# Autodesk Inventor assembly: frEonV2-AF
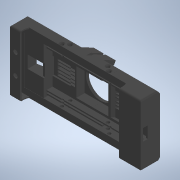
[picture p0: Inventor's stored thumbnail of the model, 180x180]
Saved by Autodesk Inventor 2020 (Build 240168000, 168)
## iProperties
Created: 2021-10-12
Part Number: frEonV2-AF
Document SubType Name: Assembly
Designer: khonsu
Author: khonsu
## Documents named in this file (5)
- D:\CAD\leeco-freon\V2\frEonV2-AF.iam
- D:\CAD\leeco-freon\V2\printed parts\left-AF.ipt
- D:\CAD\leeco-freon\V2\printed parts\right-noEONpcb-AF.ipt
- D:\CAD\leeco-freon\V2\printed parts\middle\IR-less\28DEG-CFPC-integrated.ipt
- D:\CAD\leeco-freon\V2\printed parts\middle\IR-less\bottom.ipt
## Components (4 placed, 4 different names)
1. left-AF:1 — Flush:1, Mate:1, Flush:2, Mate:3, Mate:4, Flush:3, Mate:5, Mate:6
2. right-noEONpcb-AF:1 — Flush:1, Mate:1, Flush:2, Flush:4
3. 28DEG-CFPC-integrated:1 — Mate:3, Mate:4, Flush:3
4. bottom:1 — Flush:4, Mate:5, Mate:6
## Relationships (9: Mate 5, Flush 4)
- Flush:1: left-AF:1 ↔ right-noEONpcb-AF:1
- Mate:1: left-AF:1 ↔ right-noEONpcb-AF:1
- Flush:2: left-AF:1 ↔ right-noEONpcb-AF:1
- Mate:3: left-AF:1 ↔ 28DEG-CFPC-integrated:1
- Mate:4: left-AF:1 ↔ 28DEG-CFPC-integrated:1
- Flush:3: left-AF:1 ↔ 28DEG-CFPC-integrated:1
- Flush:4: right-noEONpcb-AF:1 ↔ bottom:1
- Mate:5: left-AF:1 ↔ bottom:1
- Mate:6: left-AF:1 ↔ bottom:1
